# Autodesk Inventor assembly: SinnloseKiste
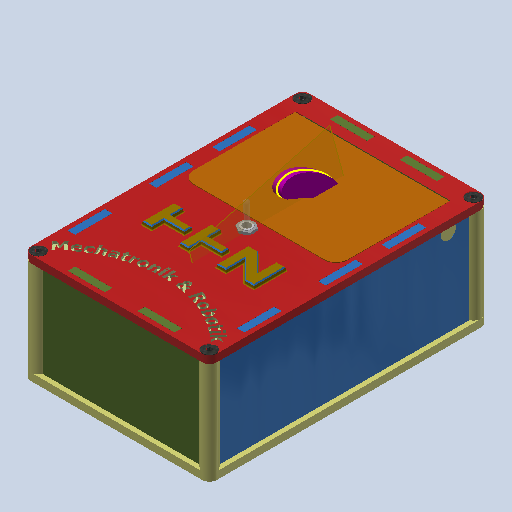
[picture p0: Inventor's stored thumbnail of the model, 512x512]
Saved by Autodesk Inventor 2025.2 (Build 292293000, 293)
## iProperties
Created: 2022-10-31
Part Number: SinnloseKiste
Material: Generisch
Description: STEP AP214
Document SubType Name: Assembly
Designer: RP
Sending System: SolidWorks 2021
Preprocessor: SwSTEP 2.0
Title: _Assembly UM_.STEP
Revision Number: ANY
## Documents named in this file (12)
- C:\Users\tino\Documents_VM\Konstruieren_CAD\Useless Box\_Useless_Box\Useless_Box.iam
- C:\Users\tino\Documents_VM\Konstruieren_CAD\Useless Box\_Useless_Box\SHort panel UM_D‚faut.ipt
- C:\Users\tino\Documents_VM\Konstruieren_CAD\Useless Box\_Useless_Box\Deckplatte.ipt
- C:\Users\tino\Documents_VM\Konstruieren_CAD\Useless Box\_Useless_Box\Klappe.ipt
- C:\Users\tino\Documents_VM\Konstruieren_CAD\Useless Box\_Useless_Box\Seitenteil_lang.ipt
- C:\Users\tino\Documents_VM\Konstruieren_CAD\Useless Box\_Useless_Box\Seitenteil_kurz.ipt
- C:\Users\tino\Documents_VM\Konstruieren_CAD\Useless Box\_Useless_Box\ISO 10642  - M4  x  12.ipt
- C:\Users\tino\Documents_VM\Konstruieren_CAD\Useless Box\_Useless_Box\ISO 10642  - M4  x  16.ipt
- C:\Users\tino\Documents_VM\Konstruieren_CAD\Useless Box\_Useless_Box\Mutter M6x0_5.ipt
- C:\Users\tino\Documents_VM\Konstruieren_CAD\Useless Box\_Useless_Box\Sicherungsscheibe M6.ipt
- C:\Users\tino\Documents_VM\Konstruieren_CAD\Useless Box\_Useless_Box\Antriebseinheit_ZSB.iam
- C:\Users\tino\Documents_VM\Konstruieren_CAD\Useless Box\_Useless_Box\Grundplatte_ZSB.iam
## Components (19 placed, 10 different names)
1. Grundplatte_ZSB:1 [sub-assembly] — Fluchtend:4, Fluchtend:5, Fluchtend:6, Einfügen:30
2. Antriebseinheit_ZSB:1 [sub-assembly]
3. DIN EN ISO 10642 M4  x  12:1 — Einfügen:30
4. DIN EN ISO 10642 M4  x  12:2
5. DIN EN ISO 10642 M4  x  12:3
6. DIN EN ISO 10642 M4  x  12:4
7. Mutter M6x0_5:3 — Einfügen:29
8. Sicherungsscheibe M6 — Einfügen:29
9. Seitenteil_lang:1
10. Seitenteil_lang:2 — Passend:34
11. Seitenteil_kurz:1
12. Seitenteil_kurz:2
13. Klappe:1 — Passend:34, Passend:39
14. Deckplatte:1 — Passend:39, Einfügen:17, Einfügen:18, Einfügen:19, Einfügen:20, Einfügen:27
15. DIN EN ISO 10642 M4  x  16:5 — Einfügen:17
16. DIN EN ISO 10642 M4  x  16:6 — Einfügen:20
17. DIN EN ISO 10642 M4  x  16:7 — Einfügen:18
18. DIN EN ISO 10642 M4  x  16:8 — Einfügen:19
19. Mutter M6x0_5:2 — Einfügen:27
## Relationships (38: Mate 20, Insert 12, Flush 4, Angle 1, Tangent 1)
- [Mate]: Grundplatte_ZSB:1 ↔ Seitenteil_lang:1
- [Mate]: Grundplatte_ZSB:1 ↔ Seitenteil_lang:1
- [Mate]: Grundplatte_ZSB:1 ↔ Seitenteil_lang:1
- [Mate]: Grundplatte_ZSB:1 ↔ Seitenteil_lang:2
- [Mate]: Grundplatte_ZSB:1 ↔ Seitenteil_lang:2
- [Mate]: Grundplatte_ZSB:1 ↔ Seitenteil_lang:2
- [Mate]: Grundplatte_ZSB:1 ↔ Seitenteil_kurz:2
- [Mate]: Grundplatte_ZSB:1 ↔ Seitenteil_kurz:2
- [Mate]: Grundplatte_ZSB:1 ↔ Seitenteil_kurz:1
- [Mate]: Grundplatte_ZSB:1 ↔ Seitenteil_kurz:2
- [Mate]: Grundplatte_ZSB:1 ↔ Seitenteil_kurz:1
- [Mate]: Grundplatte_ZSB:1 ↔ Seitenteil_kurz:1
- [Mate]: Grundplatte_ZSB:1 ↔ Seitenteil_kurz:2
- Passend:34 [Mate]: Seitenteil_lang:2 ↔ Klappe:1
- [Insert]: Grundplatte_ZSB:1 ↔ Deckplatte:1
- [Mate]: Grundplatte_ZSB:1 ↔ Deckplatte:1
- [Mate]: Antriebseinheit_ZSB:1 ↔ Deckplatte:1
- [Mate]: Grundplatte_ZSB:1 ↔ Antriebseinheit_ZSB:1
- [Angle] (0 deg): Antriebseinheit_ZSB:1
- [Tangent]: Antriebseinheit_ZSB:1 ↔ Klappe:1
- [Mate]: Antriebseinheit_ZSB:1 ↔ Klappe:1
- Passend:39 [Mate] (0.1 mm): Klappe:1 ↔ Deckplatte:1
- [Insert]: Grundplatte_ZSB:1 ↔ DIN EN ISO 10642 M4  x  12:2
- [Flush]: Grundplatte_ZSB:1 ↔ DIN EN ISO 10642 M4  x  12:1
- [Insert]: Grundplatte_ZSB:1 ↔ DIN EN ISO 10642 M4  x  12:3
- [Insert]: Grundplatte_ZSB:1 ↔ DIN EN ISO 10642 M4  x  12:4
- Einfügen:17 [Insert]: Deckplatte:1 ↔ DIN EN ISO 10642 M4  x  16:5
- Einfügen:18 [Insert]: Deckplatte:1 ↔ DIN EN ISO 10642 M4  x  16:7
- Einfügen:19 [Insert]: Deckplatte:1 ↔ DIN EN ISO 10642 M4  x  16:8
- Einfügen:20 [Insert]: Deckplatte:1 ↔ DIN EN ISO 10642 M4  x  16:6
- [Mate]: Antriebseinheit_ZSB:1 ↔ Klappe:1
- Einfügen:27 [Insert]: Deckplatte:1 ↔ Mutter M6x0_5:2
- [Insert] (0.45 mm): Antriebseinheit_ZSB:1 ↔ Mutter M6x0_5:3
- Einfügen:29 [Insert]: Mutter M6x0_5:3 ↔ Sicherungsscheibe M6
- Fluchtend:4 [Flush]: Grundplatte_ZSB:1
- Fluchtend:5 [Flush]: Grundplatte_ZSB:1
- Fluchtend:6 [Flush]: Grundplatte_ZSB:1
- Einfügen:30 [Insert]: Grundplatte_ZSB:1 ↔ DIN EN ISO 10642 M4  x  12:1
